# Autodesk Inventor assembly: Test_ASM
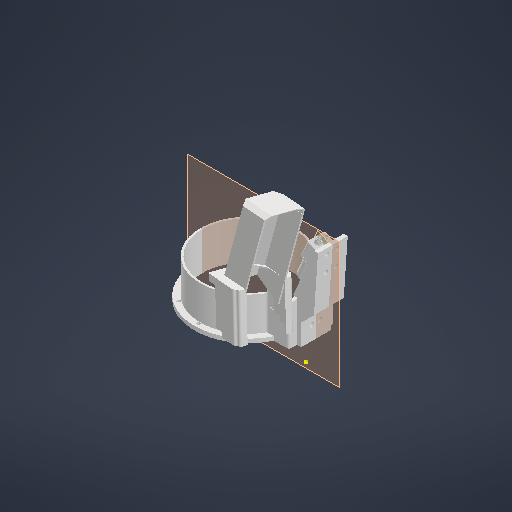
[picture p0: Inventor's stored thumbnail of the model, 512x512]
Saved by Autodesk Inventor 2026 (Build 300175000, 175)
## iProperties
Created: 2025-07-07
Part Number: Test_ASM
Document SubType Name: Assembly
Designer: Charl
Author: Charl
## Documents named in this file (4)
- E:\School\Research\Inventor\Cover\v0.3.1\Test_ASM.iam
- E:\School\Research\Inventor\Cover\v0.3.1\Holder_and_Cylinder.ipt
- E:\School\Research\Inventor\Cover\Camera\Triton2_asm.iam
- E:\School\Research\Inventor\Cover\v0.3.1\Event_Cover.ipt
## Components (3 placed, 3 different names)
1. Holder_and_Cylinder:1 — Mate:1, Mate:2
2. Triton2_asm:1 [sub-assembly] — Mate:1, Mate:2
3. Event_Cover:1
## Relationships (2: Mate 2)
- Mate:1: Holder_and_Cylinder:1 ↔ Triton2_asm:1
- Mate:2: Holder_and_Cylinder:1 ↔ Triton2_asm:1
